# Autodesk Inventor assembly: Z Axis
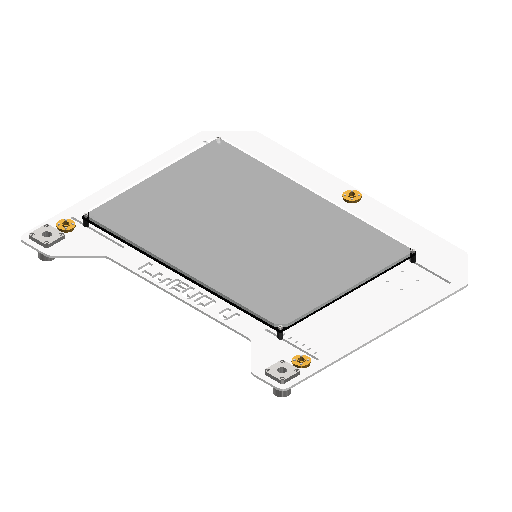
[picture p0: Inventor's stored thumbnail of the model, 512x512]
Saved by Autodesk Inventor 2023.2 (Build 272271000, 271)
## iProperties
Created: 2023-02-02
Part Number: Z Axis
Document SubType Name: Assembly
Designer: remop
Author: remop
## Documents named in this file (10)
- C:\Users\remop\OneDrive\Documents\Inventor\3D Printers\LuEVO\Mk5_FullKinematic\Z Axis v1\Z Axis.iam
- C:\Users\remop\OneDrive\Documents\Inventor\3D Printers\LuEVO\Mk5_FullKinematic\Z Axis v1\Z Axis Base.ipt
- C:\Users\remop\OneDrive\Documents\Inventor\3D Printers\LuEVO\Mk5_FullKinematic\Z Axis v2\E3D High Temperature Bed 300x200.ipt
- C:\Users\remop\OneDrive\Documents\Inventor\3D Printers\LuEVO\Mk5_FullKinematic\Z Axis v1\Z Axis Bearing.ipt
- C:\Users\remop\OneDrive\Documents\Inventor\3D Printers\LuEVO\Mk5_FullKinematic\Z Axis v1\Z Axis Nut.ipt
- C:\Users\remop\OneDrive\Documents\Inventor\3D Printers\LuEVO\Mk5_FullKinematic\Z Axis v2\Heated Bed Spacer.ipt
- C:\Users\remop\OneDrive\Documents\Inventor\3D Printers\LuEVO\Mk5_FullKinematic\Z Axis v2\Heated Bed Glass.ipt
- C:\Users\remop\OneDrive\Documents\Inventor\Content Center Files\R2023\en-US\AS 1420\AS 1420 - 1973 - M3 x 10.ipt
- C:\Users\remop\OneDrive\Documents\Inventor\Content Center Files\R2023\en-US\AS 1420\AS 1420 - 1973 - M3 x 8.ipt
- C:\Users\remop\OneDrive\Documents\Inventor\Content Center Files\R2023\en-US\AS 1112 (2)\AS 1112 - M4  Type 5.ipt
## Components (44 placed, 9 different names)
1. Z Axis Base:1 — Rigid:10, Rigid:11, Rigid:12, Rigid:13, Rigid:14, Insert:13, Insert:14, Insert:15, Insert:16, Insert:17, Insert:18, Insert:19, Insert:20, Insert:21, Insert:22, Insert:23, Insert:24, Insert:33, Insert:34, Insert:35, Insert:36, Insert:37, Insert:38, Insert:39, Insert:40, Mate:1, Flush:4
2. E3D High Temperature Bed 300x200:1 — Flush:1, Flush:2, Flush:3, Insert:1, Insert:4, Insert:6, Insert:8, Rotational:1, Rotational:2, Rotational:3, Rotational:4, Flush:4
3. Z Axis Bearing:1 — Rigid:12, Insert:25, Insert:26, Insert:27, Insert:28
4. Z Axis Bearing:2 — Rigid:11, Insert:29, Insert:30, Insert:31, Insert:32
5. Z Axis Nut:1 — Rigid:10
6. Z Axis Nut:2 — Rigid:13
7. Z Axis Nut:3 — Rigid:14
8. Heated Bed Spacer:2 — Rotational:2
9. Heated Bed Spacer:3 — Rotational:3, Mate:1
10. Heated Bed Spacer:4 — Rotational:4
11. Heated Bed Spacer:5 — Rotational:1
12. Heated Bed Glass:1 — Flush:1, Flush:2, Flush:3
13. AS 1420 - Metric M3 x 10:1 — Insert:1
14. AS 1420 - Metric M3 x 10:4 — Insert:4
15. AS 1420 - Metric M3 x 10:6 — Insert:6
16. AS 1420 - Metric M3 x 10:8 — Insert:8
17. AS 1420 - Metric M3 x 8:1 — Insert:13
18. AS 1420 - Metric M3 x 8:2 — Insert:14
19. AS 1420 - Metric M3 x 8:3 — Insert:15
20. AS 1420 - Metric M3 x 8:4 — Insert:16
21. AS 1420 - Metric M3 x 8:5 — Insert:17
22. AS 1420 - Metric M3 x 8:6 — Insert:18
23. AS 1420 - Metric M3 x 8:7 — Insert:19
24. AS 1420 - Metric M3 x 8:8 — Insert:20
25. AS 1420 - Metric M3 x 8:9 — Insert:21
26. AS 1420 - Metric M3 x 8:10 — Insert:22
27. AS 1420 - Metric M3 x 8:11 — Insert:23
28. AS 1420 - Metric M3 x 8:12 — Insert:24
29. AS 1420 - Metric M3 x 8:13 — Insert:25
30. AS 1420 - Metric M3 x 8:14 — Insert:26
31. AS 1420 - Metric M3 x 8:15 — Insert:27
32. AS 1420 - Metric M3 x 8:16 — Insert:28
33. AS 1420 - Metric M3 x 8:17 — Insert:29
34. AS 1420 - Metric M3 x 8:18 — Insert:30
35. AS 1420 - Metric M3 x 8:19 — Insert:31
36. AS 1420 - Metric M3 x 8:20 — Insert:32
37. AS 1112 (2) - Metric M4  Type 5:1 — Insert:33
38. AS 1112 (2) - Metric M4  Type 5:2 — Insert:34
39. AS 1112 (2) - Metric M4  Type 5:3 — Insert:35
40. AS 1112 (2) - Metric M4  Type 5:4 — Insert:36
41. AS 1112 (2) - Metric M4  Type 5:5 — Insert:37
42. AS 1112 (2) - Metric M4  Type 5:6 — Insert:38
43. AS 1112 (2) - Metric M4  Type 5:7 — Insert:39
44. AS 1112 (2) - Metric M4  Type 5:8 — Insert:40
## Relationships (46: Insert 32, WeldJoint 5, Flush 4, RevoluteJoint 4, Mate 1)
- Flush:1: E3D High Temperature Bed 300x200:1 ↔ Heated Bed Glass:1
- Flush:2: E3D High Temperature Bed 300x200:1 ↔ Heated Bed Glass:1
- Flush:3 (1 mm): E3D High Temperature Bed 300x200:1 ↔ Heated Bed Glass:1
- Insert:1: E3D High Temperature Bed 300x200:1 ↔ AS 1420 - Metric M3 x 10:1
- Insert:4: E3D High Temperature Bed 300x200:1 ↔ AS 1420 - Metric M3 x 10:4
- Insert:6: E3D High Temperature Bed 300x200:1 ↔ AS 1420 - Metric M3 x 10:6
- Insert:8: E3D High Temperature Bed 300x200:1 ↔ AS 1420 - Metric M3 x 10:8
- Rigid:10 [WeldJoint]: Z Axis Base:1 ↔ Z Axis Nut:1
- Rigid:11 [WeldJoint]: Z Axis Base:1 ↔ Z Axis Bearing:2
- Rigid:12 [WeldJoint]: Z Axis Base:1 ↔ Z Axis Bearing:1
- Rigid:13 [WeldJoint]: Z Axis Base:1 ↔ Z Axis Nut:2
- Rigid:14 [WeldJoint]: Z Axis Base:1 ↔ Z Axis Nut:3
- Insert:13: Z Axis Base:1 ↔ AS 1420 - Metric M3 x 8:1
- Insert:14: Z Axis Base:1 ↔ AS 1420 - Metric M3 x 8:2
- Insert:15: Z Axis Base:1 ↔ AS 1420 - Metric M3 x 8:3
- Insert:16: Z Axis Base:1 ↔ AS 1420 - Metric M3 x 8:4
- Insert:17: Z Axis Base:1 ↔ AS 1420 - Metric M3 x 8:5
- Insert:18: Z Axis Base:1 ↔ AS 1420 - Metric M3 x 8:6
- Insert:19: Z Axis Base:1 ↔ AS 1420 - Metric M3 x 8:7
- Insert:20: Z Axis Base:1 ↔ AS 1420 - Metric M3 x 8:8
- Insert:21: Z Axis Base:1 ↔ AS 1420 - Metric M3 x 8:9
- Insert:22: Z Axis Base:1 ↔ AS 1420 - Metric M3 x 8:10
- Insert:23: Z Axis Base:1 ↔ AS 1420 - Metric M3 x 8:11
- Insert:24: Z Axis Base:1 ↔ AS 1420 - Metric M3 x 8:12
- Insert:25: Z Axis Bearing:1 ↔ AS 1420 - Metric M3 x 8:13
- Insert:26: Z Axis Bearing:1 ↔ AS 1420 - Metric M3 x 8:14
- Insert:27: Z Axis Bearing:1 ↔ AS 1420 - Metric M3 x 8:15
- Insert:28: Z Axis Bearing:1 ↔ AS 1420 - Metric M3 x 8:16
- Insert:29: Z Axis Bearing:2 ↔ AS 1420 - Metric M3 x 8:17
- Insert:30: Z Axis Bearing:2 ↔ AS 1420 - Metric M3 x 8:18
- Insert:31: Z Axis Bearing:2 ↔ AS 1420 - Metric M3 x 8:19
- Insert:32: Z Axis Bearing:2 ↔ AS 1420 - Metric M3 x 8:20
- Insert:33: Z Axis Base:1 ↔ AS 1112 (2) - Metric M4  Type 5:1
- Insert:34: Z Axis Base:1 ↔ AS 1112 (2) - Metric M4  Type 5:2
- Insert:35: Z Axis Base:1 ↔ AS 1112 (2) - Metric M4  Type 5:3
- Insert:36: Z Axis Base:1 ↔ AS 1112 (2) - Metric M4  Type 5:4
- Insert:37: Z Axis Base:1 ↔ AS 1112 (2) - Metric M4  Type 5:5
- Insert:38: Z Axis Base:1 ↔ AS 1112 (2) - Metric M4  Type 5:6
- Insert:39: Z Axis Base:1 ↔ AS 1112 (2) - Metric M4  Type 5:7
- Insert:40: Z Axis Base:1 ↔ AS 1112 (2) - Metric M4  Type 5:8
- Rotational:1 [RevoluteJoint]: E3D High Temperature Bed 300x200:1 ↔ Heated Bed Spacer:5
- Rotational:2 [RevoluteJoint]: E3D High Temperature Bed 300x200:1 ↔ Heated Bed Spacer:2
- Rotational:3 [RevoluteJoint]: E3D High Temperature Bed 300x200:1 ↔ Heated Bed Spacer:3
- Rotational:4 [RevoluteJoint]: E3D High Temperature Bed 300x200:1 ↔ Heated Bed Spacer:4
- Mate:1: Z Axis Base:1 ↔ Heated Bed Spacer:3
- Flush:4 (52 mm): Z Axis Base:1 ↔ E3D High Temperature Bed 300x200:1
